# Autodesk Inventor assembly: Assembly1
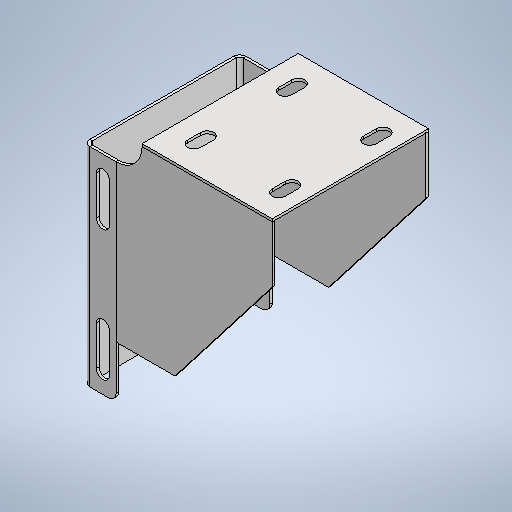
[picture p0: Inventor's stored thumbnail of the model, 512x512]
Saved by Autodesk Inventor 2025.1 (Build 291241020, 241B)
## iProperties
Created: 2024-09-16
Part Number: Assembly1
Document SubType Name: Assembly
Designer: user
Author: user
## Documents named in this file (4)
- C:\Users\user\YandexDisk-badmisterfox\домашниий пк\Inventor\BSH_Beshkino_bio_tank\Assembly1.iam
- C:\Users\user\YandexDisk-badmisterfox\домашниий пк\Inventor\BSH_Beshkino_bio_tank\TRM 026 right board damper.ipt
- C:\Users\user\YandexDisk-badmisterfox\домашниий пк\Inventor\BSH_Beshkino_bio_tank\TRM 034 motor pillar.ipt
- C:\Users\user\YandexDisk-badmisterfox\домашниий пк\Inventor\BSH_Beshkino_bio_tank\TRM 035 motor pillar 2.ipt
## Components (4 placed, 3 different names)
1. TRM 026 right board damper:1
2. TRM 034 motor pillar:1
3. TRM 034 motor pillar:2
4. TRM 035 motor pillar 2:1
## Relationships (3: WeldJoint 3)
- [WeldJoint]: TRM 026 right board damper:1 ↔ TRM 034 motor pillar:1
- [WeldJoint]: TRM 026 right board damper:1 ↔ TRM 034 motor pillar:2
- [WeldJoint]: TRM 034 motor pillar:2 ↔ TRM 035 motor pillar 2:1
